# Autodesk Inventor assembly: driver_unit_1
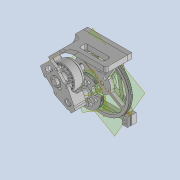
[picture p0: Inventor's stored thumbnail of the model, 180x180]
Saved by Autodesk Inventor 2020 (Build 240168000, 168)
## iProperties
Created: 2021-08-05
Part Number: driver_unit_1
Document SubType Name: Assembly
Designer: Shuang Peng
Author: Shuang Peng
## Documents named in this file (8)
- D:\projects-3\torque fb tip\hardware\tip_2\driver_unit_2\driver_unit_1.iam
- D:\projects-3\torque fb tip\hardware\tip_2\driver_unit_2\driver_wheel_1.ipt
- D:\projects-3\torque fb tip\hardware\tip_2\driver_unit_2\drv_stand_1.ipt
- D:\projects-3\torque fb tip\hardware\tip_2\mot_27_ass.iam
- D:\projects-3\torque fb tip\hardware\tip_2\tendon_wh_1_mod.ipt
- D:\projects-3\torque fb tip\hardware\tip_2\tendon_wh_3.ipt
- D:\projects-3\torque fb tip\hardware\tip_2\mot_holder_1.ipt
- D:\projects-3\torque fb tip\hardware\tip_2\mot_holder_2.ipt
## Components (7 placed, 7 different names)
1. driver_wheel_1:1 — Insert:8
2. drv_stand_1:1 — Angle:1, Flush:3, Insert:7, Insert:8
3. mot_27_ass:1 [sub-assembly] — Insert:1, Insert:2, Insert:3, Insert:4
4. tendon_wh_1_mod:1 — Insert:3, Insert:4
5. tendon_wh_3:1 — Insert:5
6. mot_holder_1:1 — Insert:1, Insert:2, Insert:5, Angle:1, Flush:4
7. mot_holder_2:1 — Flush:3, Flush:4, Insert:7
## Relationships (10: Insert 7, Flush 2, Angle 1)
- Insert:1: mot_27_ass:1 ↔ mot_holder_1:1
- Insert:2: mot_27_ass:1 ↔ mot_holder_1:1
- Insert:3: mot_27_ass:1 ↔ tendon_wh_1_mod:1
- Insert:4: mot_27_ass:1 ↔ tendon_wh_1_mod:1
- Insert:5: tendon_wh_3:1 ↔ mot_holder_1:1
- Angle:1 (-45 deg): drv_stand_1:1 ↔ mot_holder_1:1
- Flush:3: drv_stand_1:1 ↔ mot_holder_2:1
- Flush:4: mot_holder_1:1 ↔ mot_holder_2:1
- Insert:7: drv_stand_1:1 ↔ mot_holder_2:1
- Insert:8: driver_wheel_1:1 ↔ drv_stand_1:1
